# Autodesk Inventor assembly: nc_omuni_2
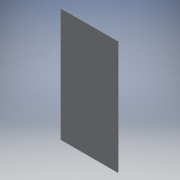
[picture p0: Inventor's stored thumbnail of the model, 180x180]
Saved by Autodesk Inventor 2019 (Build 230136000, 136)
## iProperties
Created: 2022-03-17
Part Number: nc_omuni_2
Material: 一般
Document SubType Name: Assembly
Designer: yuta
Author: yuta
## Documents named in this file (3)
- C:\Users\yuta\Documents\NHK\nc_omuni_2.iam
- C:\Users\yuta\Documents\NHK\NC.port.ipt
- C:\Users\yuta\Downloads\オムニホイール\オムニホイール\ホイールユニット_側板1.ipt
## Components (2 placed, 2 different names)
1. NC.port:1 — メイト:1, フラッシュ:1, フラッシュ:2
2. ホイールユニット_側板1:1 — メイト:1, フラッシュ:1, フラッシュ:2
## Relationships (3: Flush 2, Mate 1)
- メイト:1 [Mate]: NC.port:1 ↔ ホイールユニット_側板1:1
- フラッシュ:1 [Flush] (6 mm): NC.port:1 ↔ ホイールユニット_側板1:1
- フラッシュ:2 [Flush] (6 mm): NC.port:1 ↔ ホイールユニット_側板1:1
